# Autodesk Inventor assembly: rackRail
Saved by Autodesk Inventor 2013 (Build 170138000, 138)
## iProperties
Created: 2013-05-06
Part Number: rackRail
Document SubType Name: Assembly
Designer: istvan.burbank
Author: istvan.burbank
## Documents named in this file (7)
- C:\Users\istvan.burbank\Documents\GitHub\Crown-Fire\CAD\Frame\Table\rackRail.iam
- C:\Users\istvan.burbank\Documents\GitHub\Crown-Fire\CAD\GantryMount\rack.ipt
- C:\Users\istvan.burbank\Documents\GitHub\Crown-Fire\CAD\GantryMount\cChannel.ipt
- C:\Users\istvan.burbank\Documents\GitHub\Crown-Fire\CAD\Templates\cChannel2x1.ipt
- C:\Users\istvan.burbank\Documents\GitHub\Crown-Fire\CAD\GantryMount\y-vee-track.ipt
- C:\Users\istvan.burbank\Documents\GitHub\Crown-Fire\CAD\Templates\vee-track.ipt
- C:\Users\istvan.burbank\Documents\GitHub\Crown-Fire\CAD\GantryMount\veeTrackMount.ipt
## Components (4 placed, 4 different names)
1. rack:1
2. cChannel:1
3. y-vee-track:1
4. veeTrackMount:1
## Relationships (9: Mate 5, Flush 4)
- [Mate]: rack:1 ↔ cChannel:1
- [Flush] (6.35 mm): rack:1 ↔ cChannel:1
- [Mate]: cChannel:1 ↔ veeTrackMount:1
- [Mate]: cChannel:1 ↔ veeTrackMount:1
- [Flush]: cChannel:1 ↔ veeTrackMount:1
- [Mate]: y-vee-track:1 ↔ veeTrackMount:1
- [Flush]: y-vee-track:1 ↔ veeTrackMount:1
- [Mate]: y-vee-track:1 ↔ veeTrackMount:1
- [Flush]: rack:1 ↔ cChannel:1
